# Autodesk Inventor assembly: Assembly_XY_stage_with_motors_v3
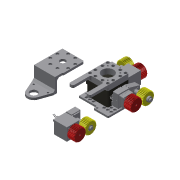
[picture p0: Inventor's stored thumbnail of the model, 180x180]
Saved by Autodesk Inventor 2019.4 (Build 234330000, 330)
## iProperties
Created: 2021-02-08
Part Number: Assembly_XY_stage_with_motors_v3
Document SubType Name: Assembly
Designer: diederichbenedict
Author: diederichbenedict
## Documents named in this file (8)
- C:\Users\diederichbenedict\Dropbox\Dokumente\Promotion\PROJECTS\UC2\02_CAD\INVENTOR\uc2_v3\cellstrom\Assembly_XY_stage_with_motors_v3.iam
- C:\Users\diederichbenedict\Dropbox\Dokumente\Promotion\PROJECTS\UC2\02_CAD\INVENTOR\uc2_v3\cellstrom\00_XY_stage-CHUO_SEIKI_LD-647-R1.iam
- C:\Users\diederichbenedict\Dropbox\Dokumente\Promotion\PROJECTS\UC2\02_CAD\INVENTOR\uc2_v3\cellstrom\cellSTORM_UC2_motorized_micrometer.iam
- C:\Users\diederichbenedict\Dropbox\Dokumente\Promotion\PROJECTS\UC2\02_CAD\INVENTOR\uc2_v3\cellstrom\30_XY_Sample_arm_v3.ipt
- C:\Users\diederichbenedict\Dropbox\Dokumente\Promotion\PROJECTS\UC2\02_CAD\INVENTOR\uc2_v3\cellstrom\cellSTORM_UC2_Laser_base.ipt
- C:\Users\diederichbenedict\Dropbox\Dokumente\Promotion\PROJECTS\UC2\02_CAD\INVENTOR\uc2_v3\cellSTORM_UC2_motorized_xystage_spacer.ipt
- C:\Users\diederichbenedict\Dropbox\Dokumente\Promotion\PROJECTS\UC2\02_CAD\INVENTOR\uc2_v3\cellstrom\cellSTORM_UC2_Sample_arm_ptycho.ipt
- C:\Users\diederichbenedict\Dropbox\Dokumente\Promotion\PROJECTS\UC2\02_CAD\INVENTOR\uc2_v3\Assembly_Nema_Motor_attachement_for_XYstage.iam
## Components (8 placed, 7 different names)
1. 00_XY_stage-CHUO_SEIKI_LD-647-R1:1 [sub-assembly] — Insert:2, Mate:3
2. cellSTORM_UC2_motorized_micrometer:1 [sub-assembly]
3. cellSTORM_UC2_motorized_micrometer:2 [sub-assembly]
4. 30_XY_Sample_arm_v3:1 — Flush:1, Flush:2
5. cellSTORM_UC2_Laser_base:1 — Insert:2, Flush:3
6. cellSTORM_UC2_motorized_xystage_spacer:1 — Flush:1, Flush:2
7. cellSTORM_UC2_Sample_arm_ptycho:1
8. Assembly_Nema_Motor_attachement_for_XYstage:1 [sub-assembly] — Mate:3, Flush:3
## Relationships (9: Mate 3, Flush 3, Insert 2, Angle 1)
- [Mate]: 00_XY_stage-CHUO_SEIKI_LD-647-R1:1 ↔ cellSTORM_UC2_motorized_micrometer:1
- [Mate]: 00_XY_stage-CHUO_SEIKI_LD-647-R1:1 ↔ cellSTORM_UC2_motorized_micrometer:2
- [Insert]: 00_XY_stage-CHUO_SEIKI_LD-647-R1:1 ↔ 30_XY_Sample_arm_v3:1
- [Angle] (0 deg): 00_XY_stage-CHUO_SEIKI_LD-647-R1:1 ↔ cellSTORM_UC2_Laser_base:1
- Insert:2: 00_XY_stage-CHUO_SEIKI_LD-647-R1:1 ↔ cellSTORM_UC2_Laser_base:1
- Flush:1: 30_XY_Sample_arm_v3:1 ↔ cellSTORM_UC2_motorized_xystage_spacer:1
- Flush:2: 30_XY_Sample_arm_v3:1 ↔ cellSTORM_UC2_motorized_xystage_spacer:1
- Mate:3: 00_XY_stage-CHUO_SEIKI_LD-647-R1:1 ↔ Assembly_Nema_Motor_attachement_for_XYstage:1
- Flush:3 (10 mm): cellSTORM_UC2_Laser_base:1 ↔ Assembly_Nema_Motor_attachement_for_XYstage:1
